# Autodesk Inventor assembly: Flutschlüssel Verriegelung
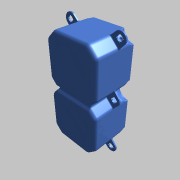
[picture p0: Inventor's stored thumbnail of the model, 180x180]
Saved by Autodesk Inventor 2015 (Build 190159000, 159)
## iProperties
Created: 2016-11-08
Part Number: Flutschlüssel Verriegelung
Project: Neuer Ordner
Document SubType Name: Assembly
Designer: Gruber
RuleStatus: InUse
AfterDocSave0: file://Projektnummer
And.-Index: 0
Dateiname: Flutschlüssel Verriegelung
Author: Gruber
## Documents named in this file (4)
- C:\Users\Seelenernter\Desktop\Neuer Ordner\Flutschlüssel Verriegelung.iam
- C:\Users\Seelenernter\Desktop\Neuer Ordner\Ponton_flutschraube.ipt
- C:\Users\Seelenernter\Desktop\Neuer Ordner\Flutschraube.ipt
- C:\Users\Seelenernter\Desktop\Neuer Ordner\Flutschlüssel.ipt
## Components (3 placed, 3 different names)
1. Ponton_flutschraube:1 — Einfügen:1, Fluchtend:1, Fluchtend:2, Winkel:3, Fluchtend:3, Winkel:4
2. Flutschraube:1 — Einfügen:1, Passend:1, Passend:2, Passend:3, Winkel:4
3. Flutschlüssel:1 — Passend:1, Passend:2, Passend:3
## Relationships (13: Mate 7, Flush 3, Angle 2, Insert 1)
- Einfügen:1 [Insert]: Ponton_flutschraube:1 ↔ Flutschraube:1
- Passend:1 [Mate]: Flutschraube:1 ↔ Flutschlüssel:1
- Passend:2 [Mate] (1 mm): Flutschraube:1 ↔ Flutschlüssel:1
- Passend:3 [Mate] (1 mm): Flutschraube:1 ↔ Flutschlüssel:1
- Fluchtend:1 [Flush]: Ponton_flutschraube:1
- Fluchtend:2 [Flush]: Ponton_flutschraube:1
- Passend:4 [Mate]
- Passend:5 [Mate]
- Passend:6 [Mate]
- Winkel:3 [Angle] (270 deg): Ponton_flutschraube:1
- Passend:7 [Mate]
- Fluchtend:3 [Flush]: Ponton_flutschraube:1
- Winkel:4 [Angle] (0 deg): Ponton_flutschraube:1 ↔ Flutschraube:1
